# Autodesk Inventor assembly: Cover Optical Camera Only
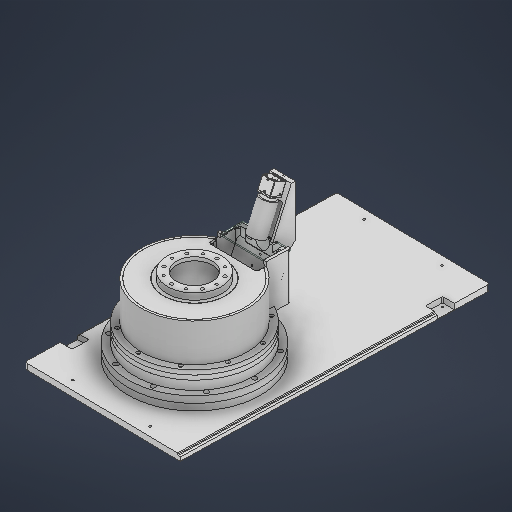
[picture p0: Inventor's stored thumbnail of the model, 512x512]
Saved by Autodesk Inventor 2025 (Build 290162000, 162)
## iProperties
Created: 2025-02-04
Part Number: Cover Optical Camera Only
Document SubType Name: Assembly
Designer: mayhe
Author: mayhe
## Documents named in this file (15)
- C:\Users\mayhe\OneDrive\Documents\GitHub\In-situ-monitoring-of-powder-bed-fusion-additive-manufacturing\system_development\Mithril\v0.2\Model\Cover Optical Camera Only.iam
- C:\Users\mayhe\OneDrive\Documents\GitHub\In-situ-monitoring-of-powder-bed-fusion-additive-manufacturing\system_development\Mithril\v0.2\Model\Cover (Optical Camera).ipt
- C:\Users\mayhe\OneDrive\Documents\GitHub\In-situ-monitoring-of-powder-bed-fusion-additive-manufacturing\system_development\Mithril\v0.2\Model\300mm Housing 1.ipt
- C:\Users\mayhe\OneDrive\Documents\GitHub\In-situ-monitoring-of-powder-bed-fusion-additive-manufacturing\system_development\Mithril\v0.2\Model\Cylinder Spacer Optical Camera.ipt
- C:\Users\mayhe\OneDrive\Documents\GitHub\In-situ-monitoring-of-powder-bed-fusion-additive-manufacturing\system_development\Mithril\v0.2\Model\Cylinder Segment\Cylinder Slidey Bit Housings\Cylinder Slidey Bit Housing Camera only v0.2.ipt
- C:\Users\mayhe\OneDrive\Documents\GitHub\In-situ-monitoring-of-powder-bed-fusion-additive-manufacturing\system_development\Mithril\v0.2\Model\300mm housing 2 Camera.ipt
- C:\Users\mayhe\OneDrive\Documents\GitHub\In-situ-monitoring-of-powder-bed-fusion-additive-manufacturing\system_development\Mithril\v0.2\Model\Cylinder Segment\Cylinder Segment  Camera only v0.2.ipt
- C:\Users\mayhe\OneDrive\Documents\GitHub\In-situ-monitoring-of-powder-bed-fusion-additive-manufacturing\system_development\Mithril\v0.2\Model\Camera Bracket.ipt
- C:\Users\mayhe\OneDrive\Documents\GitHub\In-situ-monitoring-of-powder-bed-fusion-additive-manufacturing\system_development\Mithril\v0.2\Model\flircamera+lens.ipt
- C:\Users\mayhe\OneDrive\Documents\GitHub\In-situ-monitoring-of-powder-bed-fusion-additive-manufacturing\system_development\Mithril\v0.2\Model\Cover^2 No magnets.ipt
- C:\Users\mayhe\OneDrive\Documents\GitHub\In-situ-monitoring-of-powder-bed-fusion-additive-manufacturing\system_development\Mithril\v0.2\Model\Cylinder Segment\Cylinder Segment Camera Only\C .Replace - Face.ipt
- C:\Users\mayhe\OneDrive\Documents\GitHub\In-situ-monitoring-of-powder-bed-fusion-additive-manufacturing\system_development\Mithril\v0.2\Model\Cylinder Segment\Cylinder Segment Camera Only.ipt
- C:\Users\mayhe\OneDrive\Documents\GitHub\In-situ-monitoring-of-powder-bed-fusion-additive-manufacturing\system_development\Mithril\v0.2\Model\Cylinder Segment\Cylinder Segment Camera Only\C .Replace - 10.ipt
- C:\Users\mayhe\OneDrive\Documents\GitHub\In-situ-monitoring-of-powder-bed-fusion-additive-manufacturing\system_development\Mithril\v0.2\Model\Cylinder Segment Holder.ipt
- C:\Users\mayhe\OneDrive\Documents\GitHub\In-situ-monitoring-of-powder-bed-fusion-additive-manufacturing\system_development\Mithril\v0.2\Model\Welding Glass.ipt
## Components (13 placed, 13 different names)
1. Cover (Optical Camera):1 — Rotational:1, Mate:1
2. 300mm Housing 1:1 — Rotational:1, Mate:1, Rotational:2, Mate:2
3. 300mm housing 2 Camera:1 — Rotational:2, Mate:2, Rotational:3, Mate:3
4. Cylinder Spacer Optical Camera:2 — Rotational:3, Mate:3, Rotational:4, Mate:4
5. Cylinder Segment  Camera only v0.2:1 — Rotational:4, Mate:4, Rotational:5, Mate:5, Mate:9, Cylindrical:1, Cylindrical:3, Mate:10
6. Cylinder Slidey Bit Housing Camera only v0.2:1 — Rotational:5, Mate:5, Mate:6, Mate:7, Mate:11, Mate:13
7. Camera Bracket:1 — Mate:6, Mate:7, Rotational:6, Mate:8, Mate:12
8. flircamera+lens:1 — Rotational:6, Mate:8
9. Cover^2 No magnets:1 — Mate:9
10. C .Replace - Face:1 — Cylindrical:2
11. C .Replace - 10:2 — Cylindrical:1, Cylindrical:2
12. Cylinder Segment Holder:1 — Cylindrical:3, Mate:10
13. Welding Glass:1 — Mate:11, Mate:12, Mate:13
## Relationships (23: Mate 13, RevoluteJoint 6, CylindricalJoint 3, Flush 1)
- Flush:3 (128.5875 mm)
- Rotational:1 [RevoluteJoint]: Cover (Optical Camera):1 ↔ 300mm Housing 1:1
- Mate:1: Cover (Optical Camera):1 ↔ 300mm Housing 1:1
- Rotational:2 [RevoluteJoint]: 300mm Housing 1:1 ↔ 300mm housing 2 Camera:1
- Mate:2: 300mm Housing 1:1 ↔ 300mm housing 2 Camera:1
- Rotational:3 [RevoluteJoint]: 300mm housing 2 Camera:1 ↔ Cylinder Spacer Optical Camera:2
- Mate:3: 300mm housing 2 Camera:1 ↔ Cylinder Spacer Optical Camera:2
- Rotational:4 [RevoluteJoint]: Cylinder Spacer Optical Camera:2 ↔ Cylinder Segment  Camera only v0.2:1
- Mate:4: Cylinder Spacer Optical Camera:2 ↔ Cylinder Segment  Camera only v0.2:1
- Rotational:5 [RevoluteJoint]: Cylinder Segment  Camera only v0.2:1 ↔ Cylinder Slidey Bit Housing Camera only v0.2:1
- Mate:5: Cylinder Segment  Camera only v0.2:1 ↔ Cylinder Slidey Bit Housing Camera only v0.2:1
- Mate:6: Cylinder Slidey Bit Housing Camera only v0.2:1 ↔ Camera Bracket:1
- Mate:7: Cylinder Slidey Bit Housing Camera only v0.2:1 ↔ Camera Bracket:1
- Rotational:6 [RevoluteJoint]: Camera Bracket:1 ↔ flircamera+lens:1
- Mate:8: Camera Bracket:1 ↔ flircamera+lens:1
- Mate:9: Cylinder Segment  Camera only v0.2:1 ↔ Cover^2 No magnets:1
- Cylindrical:1: Cylinder Segment  Camera only v0.2:1 ↔ C .Replace - 10:2
- Cylindrical:2: C .Replace - Face:1 ↔ C .Replace - 10:2
- Cylindrical:3: Cylinder Segment  Camera only v0.2:1 ↔ Cylinder Segment Holder:1
- Mate:10: Cylinder Segment  Camera only v0.2:1 ↔ Cylinder Segment Holder:1
- Mate:11: Cylinder Slidey Bit Housing Camera only v0.2:1 ↔ Welding Glass:1
- Mate:12: Camera Bracket:1 ↔ Welding Glass:1
- Mate:13: Cylinder Slidey Bit Housing Camera only v0.2:1 ↔ Welding Glass:1
